# Autodesk Inventor assembly: Kit Frame Long Base2
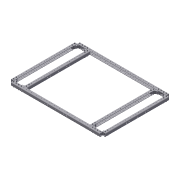
[picture p0: Inventor's stored thumbnail of the model, 180x180]
Saved by Autodesk Inventor 2011 (Build 150239000, 239)
## iProperties
Created: 2012-01-09
Part Number: Kit Frame Long Base2
Document SubType Name: Assembly
Designer: Nemo
Author: Nemo
## Documents named in this file (5)
- H:\Nemo\Documents\Robotics\COTS Parts\Kit Frame\Kit Frame Wide Base.iam
- H:\Nemo\Documents\Robotics\COTS Parts\Kit Frame\C Channel.ipt
- H:\Nemo\Documents\Robotics\COTS Parts\Kit Frame\CornerConnectAssyLeft.iam
- H:\Nemo\Documents\Robotics\COTS Parts\Kit Frame\CornerConnectAssyRight.iam
- H:\Nemo\Documents\Robotics\COTS Parts\Kit Frame\C Channel Short for Wide Base.ipt
## Components (14 placed, 4 different names)
1. C Channel:1 — Flush:1, Flush:2, Mate:1, Mate:2, Flush:3, Flush:4, Mate:4, Flush:5, Mate:8, Insert:3, Mate:18, Flush:7, Mate:24, Mate:27, Mate:28, Insert:17
2. C Channel:2 — Mate:2, Flush:3, Insert:1, Mate:14, Mate:23, Flush:6, Insert:12, Mate:25, Insert:15
3. C Channel Short for Wide Base:3 — Flush:4, Mate:4, Mate:15, Mate:29
4. C Channel Short for Wide Base:1 — Flush:5, Mate:8, Mate:19, Insert:14
5. CornerConnectAssyLeft:1 [sub-assembly] — Insert:17, Mate:29
6. CornerConnectAssyRight:1 [sub-assembly] — Insert:1, Mate:14, Mate:15
7. CornerConnectAssyLeft:2 [sub-assembly] — Insert:16, Mate:28
8. CornerConnectAssyRight:2 [sub-assembly] — Insert:10, Mate:27
9. CornerConnectAssyLeft:3 [sub-assembly] — Insert:15, Mate:26
10. CornerConnectAssyRight:3 [sub-assembly] — Insert:3, Mate:18, Mate:19
11. CornerConnectAssyLeft:4 [sub-assembly] — Insert:14, Mate:25
12. CornerConnectAssyRight:4 [sub-assembly] — Insert:12, Insert:13
13. C Channel Short for Wide Base:4 — Flush:7, Mate:24, Insert:13, Insert:16
14. C Channel Short for Wide Base:5 — Mate:23, Flush:6, Insert:10, Mate:26
## Relationships (31: Mate 15, Insert 9, Flush 7)
- Flush:1 (-342.9 mm): C Channel:1
- Flush:2: C Channel:1
- Mate:1 (87.63 mm): C Channel:1
- Mate:2: C Channel:1 ↔ C Channel:2
- Flush:3: C Channel:1 ↔ C Channel:2
- Flush:4: C Channel:1 ↔ C Channel Short for Wide Base:3
- Mate:4: C Channel:1 ↔ C Channel Short for Wide Base:3
- Flush:5: C Channel:1 ↔ C Channel Short for Wide Base:1
- Mate:8: C Channel:1 ↔ C Channel Short for Wide Base:1
- Insert:1: C Channel:2 ↔ CornerConnectAssyRight:1
- Mate:14: C Channel:2 ↔ CornerConnectAssyRight:1
- Mate:15: C Channel Short for Wide Base:3 ↔ CornerConnectAssyRight:1
- Insert:3: C Channel:1 ↔ CornerConnectAssyRight:3
- Mate:18: C Channel:1 ↔ CornerConnectAssyRight:3
- Mate:19: C Channel Short for Wide Base:1 ↔ CornerConnectAssyRight:3
- Mate:23: C Channel:2 ↔ C Channel Short for Wide Base:5
- Flush:6: C Channel:2 ↔ C Channel Short for Wide Base:5
- Insert:10: CornerConnectAssyRight:2 ↔ C Channel Short for Wide Base:5
- Flush:7: C Channel:1 ↔ C Channel Short for Wide Base:4
- Mate:24: C Channel:1 ↔ C Channel Short for Wide Base:4
- Insert:12: C Channel:2 ↔ CornerConnectAssyRight:4
- Insert:13: CornerConnectAssyRight:4 ↔ C Channel Short for Wide Base:4
- Insert:14: C Channel Short for Wide Base:1 ↔ CornerConnectAssyLeft:4
- Mate:25: C Channel:2 ↔ CornerConnectAssyLeft:4
- Insert:15: C Channel:2 ↔ CornerConnectAssyLeft:3
- Mate:26: CornerConnectAssyLeft:3 ↔ C Channel Short for Wide Base:5
- Mate:27: C Channel:1 ↔ CornerConnectAssyRight:2
- Insert:16: CornerConnectAssyLeft:2 ↔ C Channel Short for Wide Base:4
- Mate:28: C Channel:1 ↔ CornerConnectAssyLeft:2
- Insert:17: C Channel:1 ↔ CornerConnectAssyLeft:1
- Mate:29: C Channel Short for Wide Base:3 ↔ CornerConnectAssyLeft:1
